# Autodesk Inventor assembly: mesoSPIM_Steinmeyer_XYZ_stages
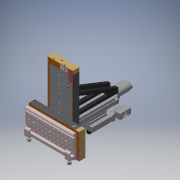
[picture p0: Inventor's stored thumbnail of the model, 180x180]
Saved by Autodesk Inventor 2019 (Build 230136000, 136)
## iProperties
Created: 2018-09-27
Part Number: mesoSPIM_Steinmeyer_XYZ_stages
Document SubType Name: Assembly
Designer: voigt
Author: voigt
## Documents named in this file (11)
- J:\Microscope_Design\CAD_Files\mesoSPIM_design_V5.2\mesoSPIM\sample_stages\mesoSPIM_Steinmeyer_XY_M406.iam
- J:\Microscope_Design\CAD_Files\mesoSPIM_design_V5.2\library\Steinmeyer_Mechatronik\PMT160-100-DCR.ipt
- J:\Microscope_Design\CAD_Files\mesoSPIM_design_V5.2\library\Steinmeyer_Mechatronik\PMT160-200-DCR.ipt
- J:\Microscope_Design\CAD_Files\mesoSPIM_design_V5.2\library\Thorlabs\accessoires\VB01_M_90deg_Bracket.ipt
- J:\Microscope_Design\CAD_Files\mesoSPIM_design_V5.2\library\Qioptiq\X95_carriers\X95_300mm_carrier\X95_300mm_Carrier.iam
- J:\Microscope_Design\CAD_Files\mesoSPIM_design_V5.2\mesoSPIM\detection_path\components\X95carrier-to-M605-adapter-V1.ipt
- J:\Microscope_Design\CAD_Files\mesoSPIM_design_V5.2\library\Physik_Instrumente\M-406-4PD-simplified.ipt
- J:\Microscope_Design\CAD_Files\mesoSPIM_design_V5.2\mesoSPIM\sample_stages\M-061-to-M-406-Adapter.ipt
- J:\Microscope_Design\CAD_Files\mesoSPIM_design_V5.2\library\Physik_Instrumente\M-061.PD-simplified.ipt
- J:\Microscope_Design\CAD_Files\mesoSPIM_design_V5.2\mesoSPIM\sample_stages\M-061-Adapter.ipt
- J:\Microscope_Design\CAD_Files\mesoSPIM_design_V5.2\library\Thorlabs\posts\post_mounts\PH50_M-Step.ipt
## Components (11 placed, 10 different names)
1. PMT160-100-DCR:1 — Mate:11, Mate:12, Mate:13, Mate:23, Mate:24, Mate:25
2. PMT160-200-DCR:1 — Mate:4, Mate:5, Angle:1, Mate:6, Mate:7, Mate:23, Mate:24, Mate:25
3. VB01_M_90deg_Bracket:1 — Mate:4, Mate:5, Angle:1, Flush:1, Angle:2, Mate:40
4. VB01_M_90deg_Bracket:2 — Mate:6, Mate:7, Flush:1, Mate:26, Mate:39
5. X95_300mm_Carrier:1 [sub-assembly] — Mate:11, Mate:12, Mate:13
6. X95carrier-to-M605-adapter-V1:1 — Mate:26, Mate:27, Mate:28, Mate:29, Angle:2, Mate:39, Mate:40
7. M-406-4PD-simplified:1 — Mate:27, Mate:28, Mate:29, Mate:30, Mate:31, Mate:32
8. M-061-to-M-406-Adapter:1 — Mate:30, Mate:31, Mate:32, Mate:33, Mate:34, Mate:35
9. M-061.PD-simplified:1 — Mate:33, Mate:34, Mate:35, Mate:36, Mate:37, Mate:38
10. M-061-Adapter:1 — Mate:36, Mate:37, Mate:38, Mate:41, Mate:42
11. PH50_M-Step:1 — Mate:41, Mate:42
## Relationships (30: Mate 27, Angle 2, Flush 1)
- Mate:4: PMT160-200-DCR:1 ↔ VB01_M_90deg_Bracket:1
- Mate:5: PMT160-200-DCR:1 ↔ VB01_M_90deg_Bracket:1
- Angle:1 (90 deg): PMT160-200-DCR:1 ↔ VB01_M_90deg_Bracket:1
- Mate:6: PMT160-200-DCR:1 ↔ VB01_M_90deg_Bracket:2
- Mate:7: PMT160-200-DCR:1 ↔ VB01_M_90deg_Bracket:2
- Flush:1: VB01_M_90deg_Bracket:1 ↔ VB01_M_90deg_Bracket:2
- Mate:11: PMT160-100-DCR:1 ↔ X95_300mm_Carrier:1
- Mate:12: PMT160-100-DCR:1 ↔ X95_300mm_Carrier:1
- Mate:13: PMT160-100-DCR:1 ↔ X95_300mm_Carrier:1
- Mate:23: PMT160-100-DCR:1 ↔ PMT160-200-DCR:1
- Mate:24: PMT160-100-DCR:1 ↔ PMT160-200-DCR:1
- Mate:25: PMT160-100-DCR:1 ↔ PMT160-200-DCR:1
- Mate:26: VB01_M_90deg_Bracket:2 ↔ X95carrier-to-M605-adapter-V1:1
- Mate:27: X95carrier-to-M605-adapter-V1:1 ↔ M-406-4PD-simplified:1
- Mate:28: X95carrier-to-M605-adapter-V1:1 ↔ M-406-4PD-simplified:1
- Mate:29: X95carrier-to-M605-adapter-V1:1 ↔ M-406-4PD-simplified:1
- Mate:30: M-406-4PD-simplified:1 ↔ M-061-to-M-406-Adapter:1
- Mate:31: M-406-4PD-simplified:1 ↔ M-061-to-M-406-Adapter:1
- Mate:32: M-406-4PD-simplified:1 ↔ M-061-to-M-406-Adapter:1
- Mate:33: M-061-to-M-406-Adapter:1 ↔ M-061.PD-simplified:1
- Mate:34: M-061-to-M-406-Adapter:1 ↔ M-061.PD-simplified:1
- Mate:35: M-061-to-M-406-Adapter:1 ↔ M-061.PD-simplified:1
- Mate:36: M-061.PD-simplified:1 ↔ M-061-Adapter:1
- Mate:37: M-061.PD-simplified:1 ↔ M-061-Adapter:1
- Mate:38: M-061.PD-simplified:1 ↔ M-061-Adapter:1
- Angle:2 (0 deg): VB01_M_90deg_Bracket:1 ↔ X95carrier-to-M605-adapter-V1:1
- Mate:39: VB01_M_90deg_Bracket:2 ↔ X95carrier-to-M605-adapter-V1:1
- Mate:40: VB01_M_90deg_Bracket:1 ↔ X95carrier-to-M605-adapter-V1:1
- Mate:41: M-061-Adapter:1 ↔ PH50_M-Step:1
- Mate:42: M-061-Adapter:1 ↔ PH50_M-Step:1
